# Autodesk Inventor assembly: mechanum wheel_2
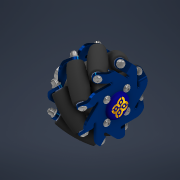
[picture p0: Inventor's stored thumbnail of the model, 180x180]
Saved by Autodesk Inventor 2021.3 (Build 253353000, 353)
## iProperties
Created: 2021-10-17
Part Number: mechanum wheel_2
Document SubType Name: Assembly
Designer: ASUS
Author: ASUS
## Documents named in this file (11)
- E:\Inventor\mecanum wheel\mechanum wheel_2.iam
- E:\Inventor\mecanum wheel\shaft.ipt
- E:\Inventor\mecanum wheel\frame.ipt
- E:\Inventor\mecanum wheel\bolt.ipt
- C:\Users\ASUS\Documents\Inventor\Content Center Files\R2021\en-US\ISO 10511\ISO 10511 - M3.ipt
- E:\Inventor\mecanum wheel\roller.ipt
- E:\Inventor\mecanum wheel\roller bracket.ipt
- E:\Inventor\mecanum wheel\roller bracket_MIR.ipt
- E:\Inventor\mecanum wheel\tutup.ipt
- E:\Inventor\mecanum wheel\tuk-tukan.ipt
- E:\Inventor\mecanum wheel\bolt_2_5mm.ipt
## Components (55 placed, 10 different names)
1. shaft:1 — Mate:1, Mate:2, Mate:3, Mate:4, Mate:5, Mate:6, Mate:7, Mate:8, Mate:29
2. frame:1 — Mate:4, Mate:5, Mate:6, Mate:15, Mate:23, Mate:30
3. frame:2 — Mate:7, Mate:8, Rigid:1, Mate:13, Mate:14, Mate:17, Mate:28
4. tuk-tukan:1 — Mate:23, Mate:24, Mate:25, Cylindrical:1, Mate:26
5. tutup:1 — Mate:28, Mate:29
6. bolt:1 — Rigid:1, Mate:24, Mate:27
7. bolt:2
8. bolt:3
9. bolt:4 — Mate:25
10. bolt:5 — Mate:16, Mate:17, Mate:31
11. roller:1 — Mate:9, Mate:10, Mate:11, Mate:12, Mate:14, Mate:15, Mate:16
12. roller bracket:1 — Mate:9, Mate:10, Mate:13
13. roller bracket_MIR:1 — Mate:11, Mate:12
14. DIN EN ISO 10511 M3:6 — Mate:30, Mate:31
15. bolt:6
16. roller:2
17. roller bracket:2
18. roller bracket_MIR:2
19. DIN EN ISO 10511 M3:7
20. bolt:7
21. roller:3
22. roller bracket:3
23. roller bracket_MIR:3
24. DIN EN ISO 10511 M3:8
25. bolt:8
26. roller:4
27. roller bracket:4
28. roller bracket_MIR:4
29. DIN EN ISO 10511 M3:9
30. bolt:10
31. roller:6
32. roller bracket:8
33. roller bracket_MIR:5
34. DIN EN ISO 10511 M3:10
35. bolt:11
36. roller:7
37. roller bracket:9
38. roller bracket_MIR:6
39. DIN EN ISO 10511 M3:11
40. bolt:12
41. roller:8
42. roller bracket:10
43. roller bracket_MIR:7
44. DIN EN ISO 10511 M3:12
45. bolt:13
46. roller:9
47. roller bracket:11
48. roller bracket_MIR:8
49. DIN EN ISO 10511 M3:13
50. bolt_2_5mm:1 — Cylindrical:1
51. bolt_2_5mm:2
52. DIN EN ISO 10511 M3:14 — Mate:26, Mate:27
53. DIN EN ISO 10511 M3:15
54. DIN EN ISO 10511 M3:16
55. DIN EN ISO 10511 M3:17
## Component patterns: (4 elements, first: bolt:1), (8 elements, first: bolt:5 + roller:1 + roller bracket:1 + roller bracket_MIR:1 + DIN EN ISO 10511 M3:6), (2 elements, first: bolt_2_5mm:1), (4 elements, first: DIN EN ISO 10511 M3:14)
## Relationships (28: Mate 26, WeldJoint 1, CylindricalJoint 1)
- Mate:1: shaft:1
- Mate:2: shaft:1
- Mate:3: shaft:1
- Mate:4: shaft:1 ↔ frame:1
- Mate:5: shaft:1 ↔ frame:1
- Mate:6: shaft:1 ↔ frame:1
- Mate:7: shaft:1 ↔ frame:2
- Mate:8: shaft:1 ↔ frame:2
- Rigid:1 [WeldJoint]: frame:2 ↔ bolt:1
- Mate:9: roller:1 ↔ roller bracket:1
- Mate:10: roller:1 ↔ roller bracket:1
- Mate:11: roller:1 ↔ roller bracket_MIR:1
- Mate:12: roller:1 ↔ roller bracket_MIR:1
- Mate:13: frame:2 ↔ roller bracket:1
- Mate:14: frame:2 ↔ roller:1
- Mate:15: frame:1 ↔ roller:1
- Mate:16: bolt:5 ↔ roller:1
- Mate:17: frame:2 ↔ bolt:5
- Mate:23: frame:1 ↔ tuk-tukan:1
- Mate:24: tuk-tukan:1 ↔ bolt:1
- Mate:25: tuk-tukan:1 ↔ bolt:4
- Cylindrical:1: tuk-tukan:1 ↔ bolt_2_5mm:1
- Mate:26: tuk-tukan:1 ↔ DIN EN ISO 10511 M3:14
- Mate:27: bolt:1 ↔ DIN EN ISO 10511 M3:14
- Mate:28: frame:2 ↔ tutup:1
- Mate:29: shaft:1 ↔ tutup:1
- Mate:30: frame:1 ↔ DIN EN ISO 10511 M3:6
- Mate:31: bolt:5 ↔ DIN EN ISO 10511 M3:6
